# Autodesk Inventor assembly: ПереПереСборка лица
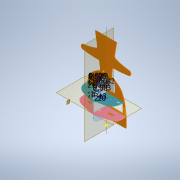
[picture p0: Inventor's stored thumbnail of the model, 180x180]
Saved by Autodesk Inventor 2020 (Build 240168000, 168)
## iProperties
Created: 2022-06-06
Part Number: ПереПереСборка лица
Document SubType Name: Assembly
Designer: Администратор
Author: Администратор
## Documents named in this file (6)
- C:\Users\air13\Documents\3D\уборка\Face 2.0 full\2\ПереПереСборка лица.iam
- C:\Users\air13\Documents\3D\уборка\Face 2.0 full\2\платформа_глаза.ipt
- C:\Users\air13\Documents\3D\уборка\Face 2.0 full\2\платформа_для_бровей.ipt
- C:\Users\air13\Documents\3D\уборка\Face 2.0 full\2\поперечная_поддержка.ipt
- C:\Users\air13\Documents\3D\уборка\Face 2.0 full\2\head_1.ipt
- C:\Users\air13\Documents\3D\уборка\Face 2.0 full\2\ard_uno_r3.ipt
## Components (6 placed, 5 different names)
1. платформа_глаза:1 — Совмещение:2, Совмещение:3, Заподлицо:3
2. платформа_для_бровей:1 — Заподлицо:1, Совмещение:4, Заподлицо:2, Совмещение:13
3. поперечная_поддержка:1 — Совмещение:1, Совмещение:3, Совмещение:4, Заподлицо:2, Заподлицо:3, Совмещение:5, Совмещение:6
4. head_1:1 — Заподлицо:4, Совмещение:5, Совмещение:6, Совмещение:7, Совмещение:8, Совмещение:9, Совмещение:10, Совмещение:11, Совмещение:12, Совмещение:13
5. ard_uno_r3:1 — Совмещение:7, Совмещение:8, Совмещение:9
6. ard_uno_r3:2 — Совмещение:10, Совмещение:11, Совмещение:12
## Relationships (17: Mate 13, Flush 4)
- Совмещение:1 [Mate]: поперечная_поддержка:1
- Заподлицо:1 [Flush]: платформа_для_бровей:1
- Совмещение:2 [Mate]: платформа_глаза:1
- Совмещение:3 [Mate]: платформа_глаза:1 ↔ поперечная_поддержка:1
- Совмещение:4 [Mate]: платформа_для_бровей:1 ↔ поперечная_поддержка:1
- Заподлицо:2 [Flush]: платформа_для_бровей:1 ↔ поперечная_поддержка:1
- Заподлицо:3 [Flush]: платформа_глаза:1 ↔ поперечная_поддержка:1
- Заподлицо:4 [Flush]: head_1:1
- Совмещение:5 [Mate]: поперечная_поддержка:1 ↔ head_1:1
- Совмещение:6 [Mate]: поперечная_поддержка:1 ↔ head_1:1
- Совмещение:7 [Mate]: head_1:1 ↔ ard_uno_r3:1
- Совмещение:8 [Mate]: head_1:1 ↔ ard_uno_r3:1
- Совмещение:9 [Mate]: head_1:1 ↔ ard_uno_r3:1
- Совмещение:10 [Mate]: head_1:1 ↔ ard_uno_r3:2
- Совмещение:11 [Mate]: head_1:1 ↔ ard_uno_r3:2
- Совмещение:12 [Mate]: head_1:1 ↔ ard_uno_r3:2
- Совмещение:13 [Mate]: платформа_для_бровей:1 ↔ head_1:1
